# Autodesk Inventor assembly: Brazo
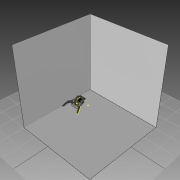
[picture p0: Inventor's stored thumbnail of the model, 180x180]
Saved by Autodesk Inventor 2015 (Build 190159000, 159)
## iProperties
Created: 2013-10-22
Part Number: Brazo
Document SubType Name: Assembly
Designer: Gregorio
Author: Gregorio
## Documents named in this file (12)
- C:\Users\Gregorio\Documents\Curso 2013-2014\Brazo Robótico\RC\Piezas Inventor\Brazo.iam
- C:\Users\Gregorio\Documents\Curso 2013-2014\Brazo Robótico\RC\Piezas Inventor\Enlace1.ipt
- C:\Users\Gregorio\Documents\Curso 2013-2014\Brazo Robótico\RC\Piezas Inventor\Enlace2.ipt
- C:\Users\Gregorio\Documents\Curso 2013-2014\Brazo Robótico\RC\Piezas Inventor\Servo.ipt
- C:\Users\Gregorio\Documents\Curso 2013-2014\Brazo Robótico\RC\Piezas Inventor\Pinza.ipt
- C:\Users\Gregorio\Documents\Curso 2013-2014\Brazo Robótico\RC\Piezas Inventor\BrazoPinza2.ipt
- C:\Users\Gregorio\Documents\Curso 2013-2014\Brazo Robótico\RC\Piezas Inventor\BrazoPinza.ipt
- C:\Users\Gregorio\Documents\Curso 2013-2014\Brazo Robótico\RC\Piezas Inventor\Enlace2Base.ipt
- C:\Users\Gregorio\Documents\Curso 2013-2014\Brazo Robótico\RC\Piezas Inventor\Servo2.ipt
- C:\Users\Gregorio\Documents\Curso 2013-2014\Brazo Robótico\RC\Piezas Inventor\BaseVentosa.ipt
- C:\Users\Gregorio\Documents\Curso 2013-2014\Brazo Robótico\RC\Piezas Inventor\SoporteVentosa.ipt
- C:\Users\Gregorio\Documents\Curso 2013-2014\Brazo Robótico\RC\Piezas Inventor\Plano.ipt
## Components (22 placed, 11 different names)
1. Servo:3 — Coincidencia:3, Ángulo:12, Insertar:27, Insertar:28
2. Pinza:1 — Insertar:5, Ángulo:5, Insertar:10, Insertar:18
3. Servo:4 — Insertar:5, Ángulo:5, Insertar:8
4. BrazoPinza2:1 — Insertar:8, Rotación:2
5. Enlace2:2 — Insertar:10, Ángulo:6, Insertar:11, Insertar:30
6. Servo:5 — Ángulo:6, Insertar:11
7. BrazoPinza:1 — Insertar:18, Rotación:2
8. Enlace1:2 — Coincidencia:1, Ángulo:9, Insertar:23
9. Enlace2Base:2 — Insertar:29
10. Servo2:2
11. Servo:7 — Coincidencia:1, Ángulo:9, Insertar:23, Insertar:30
12. Enlace1:3
13. Enlace2Base:3 — Insertar:28
14. Servo2:3
15. Servo:8 — Insertar:29
16. BaseVentosa:1 — Coincidencia:3, Ángulo:12, Insertar:27, Coincidencia:4, Coincidencia:5, Coincidencia:6, Coincidencia:7, Coincidencia:8, Coincidencia:9
17. SoporteVentosa:1 — Coincidencia:4, Coincidencia:5
18. SoporteVentosa:2 — Coincidencia:6, Coincidencia:7
19. SoporteVentosa:3 — Coincidencia:8, Coincidencia:9
20. Plano:1
21. Plano:2
22. Plano:3
## Relationships (32: Insert 15, Mate 9, Angle 7, RelateRotation 1)
- Insertar:5 (2 mm): Pinza:1 ↔ Servo:4
- Ángulo:5 [Angle] (0 deg): Pinza:1 ↔ Servo:4
- Insertar:8 (2 mm): Servo:4 ↔ BrazoPinza2:1
- Insertar:10: Pinza:1 ↔ Enlace2:2
- Ángulo:6 [Angle] (0 deg): Enlace2:2 ↔ Servo:5
- Insertar:11 (-3 mm): Enlace2:2 ↔ Servo:5
- Insertar:18 (-3 mm): Pinza:1 ↔ BrazoPinza:1
- Rotación:2 [RelateRotation] (1 ul): BrazoPinza2:1 ↔ BrazoPinza:1
- [Insert]: Enlace1:2 ↔ Enlace2Base:2
- [Insert]: Enlace2Base:2 ↔ Servo2:2
- [Angle] (0 deg): Enlace2Base:2 ↔ Servo2:2
- Coincidencia:1 [Mate]: Enlace1:2 ↔ Servo:7
- Ángulo:9 [Angle] (180 deg): Enlace1:2 ↔ Servo:7
- Insertar:23 (-2 mm): Enlace1:2 ↔ Servo:7
- [Insert]: Enlace1:3 ↔ Enlace2Base:3
- [Insert]: Enlace2Base:3 ↔ Servo2:3
- [Angle] (0 deg): Enlace2Base:3 ↔ Servo2:3
- [Mate]: Enlace1:3 ↔ Servo:8
- [Angle] (180 deg): Enlace1:3 ↔ Servo:8
- [Insert] (-2 mm): Enlace1:3 ↔ Servo:8
- Coincidencia:3 [Mate]: Servo:3 ↔ BaseVentosa:1
- Ángulo:12 [Angle] (0 deg): Servo:3 ↔ BaseVentosa:1
- Insertar:27 (-2 mm): Servo:3 ↔ BaseVentosa:1
- Insertar:28: Servo:3 ↔ Enlace2Base:3
- Insertar:29: Enlace2Base:2 ↔ Servo:8
- Insertar:30: Enlace2:2 ↔ Servo:7
- Coincidencia:4 [Mate]: BaseVentosa:1 ↔ SoporteVentosa:1
- Coincidencia:5 [Mate]: BaseVentosa:1 ↔ SoporteVentosa:1
- Coincidencia:6 [Mate]: BaseVentosa:1 ↔ SoporteVentosa:2
- Coincidencia:7 [Mate]: BaseVentosa:1 ↔ SoporteVentosa:2
- Coincidencia:8 [Mate]: BaseVentosa:1 ↔ SoporteVentosa:3
- Coincidencia:9 [Mate]: BaseVentosa:1 ↔ SoporteVentosa:3
## Named parameters: d85_d73 = 0 mm, d86_d83 = 0 mm, d87_d84 = 0 deg, d95_d94 = -2 mm, d96_d89 = 180 deg, d97_d92 = 0 mm, d98_d85_d73 = 0 mm, d99_d86_d83 = 0 mm, d100_d87_d84 = 0 deg
